# Autodesk Inventor assembly: Structure
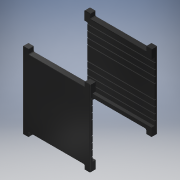
[picture p0: Inventor's stored thumbnail of the model, 180x180]
Saved by Autodesk Inventor 2018 (Build 220112000, 112)
## iProperties
Created: 2018-07-04
Part Number: Structure
Document SubType Name: Assembly
Designer: Bradley
Author: Bradley
## Documents named in this file (3)
- D:\Users\Bradley\Documents\CougsInSpace\CougSat1-Hardware\CougSat1-Structure\CADModel\Native\Structure.iam
- D:\Users\Bradley\Documents\CougsInSpace\CougSat1-Hardware\CougSat1-Structure\CADModel\Native\Structure_+Y.ipt
- D:\Users\Bradley\Documents\CougsInSpace\CougSat1-Hardware\CougSat1-Structure\CADModel\Native\Structure_-Y.ipt
## Components (2 placed, 2 different names)
1. Structure_+Y:1 — Flush:1, Flush:2, Symmetry:1, Mate:1
2. Structure_-Y:1 — Flush:3, Flush:4, Symmetry:1, Mate:1
## Relationships (6: Flush 4, Symmetry 1, Mate 1)
- Flush:1: Structure_+Y:1
- Flush:2: Structure_+Y:1
- Flush:3: Structure_-Y:1
- Flush:4: Structure_-Y:1
- Symmetry:1: Structure_+Y:1 ↔ Structure_-Y:1
- Mate:1 (-100 mm): Structure_+Y:1 ↔ Structure_-Y:1
